# Autodesk Inventor assembly: Storage System Assembly
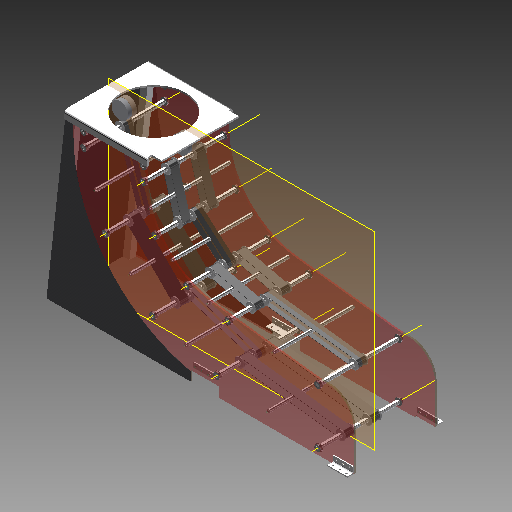
[picture p0: Inventor's stored thumbnail of the model, 512x512]
Saved by Autodesk Inventor 2019.4 (Build 234330000, 330)
## iProperties
Created: 2020-01-11
Part Number: Storage System Assembly
Document SubType Name: Assembly
Designer: admin
Mass: 9233.81 g
Surface Area: 26399.2 cm^2
Volume: 4839.78 cm^3
Density: 1.9079 g/cm^3
Author: admin
## Documents named in this file (23)
- C:\Users\Mark\Desktop\7738 Helion Engineering\7738-2020\Storage system\Storage System Assembly.iam
- C:\Users\Mark\Desktop\7738 Helion Engineering\7738-2020\Storage system\Turret Base Plate.ipt
- C:\Users\Mark\Desktop\7738 Helion Engineering\7738-2020\Storage system\Storage Side Plate.ipt
- C:\Users\Mark\Desktop\7738 Helion Engineering\7738-2020\CAD\Gearbox\F6800.ipt
- C:\Users\Mark\Desktop\7738 Helion Engineering\7738-2020\Storage system\Storage System Assembly\Design Accelerator\Synchronous Belts Transmission1.iam
- C:\Users\Mark\Desktop\7738 Helion Engineering\7738-2020\Storage system\Storage System Assembly\Design Accelerator\Synchronous Belts Transmission2.iam
- C:\Users\Mark\Desktop\7738 Helion Engineering\7738-2020\Storage system\Storage System Assembly\Design Accelerator\Synchronous Belts Transmission3.iam
- C:\Users\Mark\Desktop\7738 Helion Engineering\7738-2020\Storage system\Storage System Assembly\Design Accelerator\Synchronous Belts Transmission5.iam
- C:\Users\Mark\Desktop\7738 Helion Engineering\7738-2020\Storage system\Storage System Assembly\Design Accelerator\Synchronous Belts Transmission6.iam
- C:\Users\Mark\Desktop\7738 Helion Engineering\7738-2020\Storage system\Storage System Assembly\Design Accelerator\Synchronous Belts Transmission7.iam
- C:\Users\Mark\Desktop\7738 Helion Engineering\7738-2020\Storage system\Storage System Assembly\Design Accelerator\Synchronous Belts Transmission8.iam
- C:\Users\Mark\Desktop\7738 Helion Engineering\7738-2020\Storage system\Storage System Assembly\Design Accelerator\Synchronous Belts Transmission9.iam
- C:\Users\Mark\Desktop\7738 Helion Engineering\7738-2020\Storage system\Complaint Wheel.ipt
- C:\Users\Mark\Desktop\7738 Helion Engineering\7738-2020\Storage system\Belt Axle.ipt
- C:\Users\Mark\Desktop\7738 Helion Engineering\7738-2020\Storage system\Storage System Assembly\Design Accelerator\Synchronous Belts Transmission4.iam
- C:\Users\Mark\Desktop\7738 Helion Engineering\7738-2020\Storage system\Storage System Assembly\Design Accelerator\Synchronous Belts Transmission10.iam
- C:\Users\Mark\Desktop\7738 Helion Engineering\7738-2020\Storage system\Storage System Assembly\Design Accelerator\Synchronous Belts Transmission11.iam
- C:\Users\Mark\Desktop\7738 Helion Engineering\7738-2020\Storage system\Storage System Assembly\Design Accelerator\Synchronous Belts Transmission12.iam
- C:\Users\Mark\Desktop\7738 Helion Engineering\7738-2020\Storage system\Storage Plate Spacer.ipt
- C:\Users\Mark\Desktop\7738 Helion Engineering\7738-2020\Storage system\PC Plate Bracket.ipt
- C:\Users\Mark\Desktop\7738 Helion Engineering\7738-2020\Storage system\Turret Support Extrusion.ipt
- C:\Users\Mark\Desktop\7738 Helion Engineering\7738-2020\Storage system\Back PC Cover.ipt
- C:\Users\Mark\Desktop\7738 Helion Engineering\7738-2020\Storage system\Side CFRP Cover.ipt
## Components (70 placed, 11 different names)
1. Turret Base Plate:1 — Mate:1, Mate:3, Mate:4, Flush:1, Mate:5, Mate:8, Mate:9, Angle:1, Mate:107, Mate:108, Mate:110
2. Storage Side Plate:1 — Mate:1, Mate:7, Mate:8, Mate:10, Mate:11, Mate:12, Mate:13, Mate:14, Mate:15, Mate:16, Mate:17, Mate:18, Mate:19, Mate:20, Mate:21, Mate:22, Mate:23, Mate:24, Mate:25, Mate:26, Mate:27, Mate:28, Mate:29, Mate:30, Mate:31, Mate:32, Mate:33, Symmetry:1, Mate:75, Mate:93, Mate:94, Mate:95, Mate:96, Mate:97, Mate:98, Mate:99, Mate:100, Mate:101, Flush:4, Mate:102, Mate:105, Flush:6, Flush:7, Mate:107, Mate:111, Flush:11, Mate:114, Mate:115, Flush:12, Flush:13
3. Storage Side Plate:2 — Mate:5, Mate:7, Mate:9, Symmetry:1, Mate:41, Mate:42, Mate:43, Mate:44, Mate:45, Mate:46, Mate:47, Mate:48, Mate:49, Mate:50, Mate:51, Mate:52, Mate:53, Mate:54, Mate:55, Mate:56, Mate:57, Mate:58, Mate:59, Mate:60, Mate:61, Mate:62, Mate:63, Mate:64, Mate:85, Mate:86, Mate:87, Mate:88, Mate:89, Mate:90, Mate:91, Mate:92, Mate:103, Mate:104, Flush:5, Mate:106, Flush:8, Flush:9, Mate:109, Flush:10, Mate:113, Mate:116, Flush:14, Flush:15
4. Synchronous Belts Transmission:1 [sub-assembly] — Mate:66
5. Synchronous Belts Transmission:2 [sub-assembly]
6. Synchronous Belts Transmission:3 [sub-assembly]
7. Synchronous Belts Transmission:4 [sub-assembly]
8. Synchronous Belts Transmission:5 [sub-assembly]
9. Synchronous Belts Transmission:6 [sub-assembly]
10. Synchronous Belts Transmission:7 [sub-assembly]
11. Synchronous Belts Transmission:8 [sub-assembly]
12. F6800:11 — Mate:30, Mate:32, Mate:34
13. F6800:12 — Mate:31, Mate:33, Mate:39
14. Complaint Wheel:1 — Mate:34, Mate:35, Mate:36, Flush:3
15. Complaint Wheel:2 — Mate:35, Mate:36, Mate:40
16. Complaint Wheel:3 — Flush:3
17. Complaint Wheel:4 — Mate:39
18. Synchronous Belts Transmission:9 [sub-assembly]
19. Synchronous Belts Transmission:10 [sub-assembly]
20. Synchronous Belts Transmission:11 [sub-assembly]
21. Synchronous Belts Transmission:12 [sub-assembly]
22. Storage Plate Spacer:1 — Mate:85, Mate:93
23. Storage Plate Spacer:2 — Mate:89, Mate:100
24. Storage Plate Spacer:3 — Mate:90, Mate:99
25. Storage Plate Spacer:4 — Mate:91, Mate:98
26. Storage Plate Spacer:5 — Mate:92, Mate:97
27. Storage Plate Spacer:6 — Mate:88, Mate:96
28. Storage Plate Spacer:7 — Mate:87, Mate:95
29. Storage Plate Spacer:8 — Mate:86, Mate:94
30. PC Plate Bracket:1 — Mate:101, Flush:4, Mate:102
31. PC Plate Bracket:2 — Mate:103, Mate:104, Flush:5
32. PC Plate Bracket:3 — Mate:105, Flush:6, Flush:7
33. PC Plate Bracket:4 — Mate:106, Flush:8, Flush:9
34. Turret Support Extrusion:1 — Mate:108, Mate:109, Flush:10, Mate:112
35. Turret Support Extrusion:2 — Mate:110, Mate:111, Flush:11
36. Back PC Cover:1 — Mate:112, Mate:113, Mate:114
37. Side CFRP Cover:1 — Mate:115, Flush:12, Flush:13
38. Side CFRP Cover:2 — Mate:116, Flush:14, Flush:15
39. Belt Axle:10 — Mate:74, Mate:84
40. Belt Axle:9 — Mate:73, Mate:83
41. Belt Axle:8 — Mate:72, Mate:82
42. Belt Axle:7 — Mate:71, Mate:81
43. Belt Axle:6 — Mate:70, Mate:80
44. Belt Axle:5 — Mate:69, Mate:75
45. Belt Axle:4 — Mate:68, Mate:76
46. Belt Axle:3 — Mate:67, Mate:77
47. Belt Axle:2 — Mate:66, Mate:78
48. Belt Axle:1 — Mate:65, Mate:79
49. F6800:10 — Mate:19, Mate:25, Mate:70, Mate:80
50. F6800:9 — Mate:18, Mate:26, Mate:71, Mate:81
51. F6800:7 — Mate:16, Mate:28, Mate:73, Mate:83
52. F6800:8 — Mate:17, Mate:27, Mate:72, Mate:82
53. F6800:6 — Mate:15, Mate:29, Mate:74, Mate:84
54. F6800:5 — Mate:14, Mate:24, Mate:69
55. F6800:4 — Mate:13, Mate:23, Mate:68, Mate:76
56. F6800:3 — Mate:12, Mate:22, Mate:67, Mate:77
57. F6800:2 — Mate:11, Mate:21, Mate:78
58. F6800:1 — Mate:10, Mate:20, Mate:65, Mate:79
59. F6800:24 — Mate:52, Mate:64
60. F6800:23 — Mate:51, Mate:63
61. F6800:22 — Mate:49, Mate:61
62. F6800:21 — Mate:50, Mate:62
63. F6800:20 — Mate:48, Mate:60
64. F6800:19 — Mate:47, Mate:59
65. F6800:18 — Mate:46, Mate:57
66. F6800:17 — Mate:45, Mate:58
67. F6800:16 — Mate:44, Mate:55
68. F6800:15 — Mate:42, Mate:53
69. F6800:13 — Mate:41, Mate:54
70. F6800:14 — Mate:43, Mate:56
## Relationships (130: Mate 114, Flush 14, Angle 1, Symmetry 1)
- Mate:1: Turret Base Plate:1 ↔ Storage Side Plate:1
- Mate:3: Turret Base Plate:1
- Mate:4: Turret Base Plate:1
- Flush:1: Turret Base Plate:1
- Mate:5: Turret Base Plate:1 ↔ Storage Side Plate:2
- Mate:7: Storage Side Plate:1 ↔ Storage Side Plate:2
- Mate:8 (3 mm): Turret Base Plate:1 ↔ Storage Side Plate:1
- Mate:9 (3 mm): Turret Base Plate:1 ↔ Storage Side Plate:2
- Mate:10: Storage Side Plate:1 ↔ F6800:1
- Mate:11: Storage Side Plate:1 ↔ F6800:2
- Mate:12: Storage Side Plate:1 ↔ F6800:3
- Mate:13: Storage Side Plate:1 ↔ F6800:4
- Mate:14: Storage Side Plate:1 ↔ F6800:5
- Mate:15: Storage Side Plate:1 ↔ F6800:6
- Mate:16: Storage Side Plate:1 ↔ F6800:7
- Mate:17: Storage Side Plate:1 ↔ F6800:8
- Mate:18: Storage Side Plate:1 ↔ F6800:9
- Mate:19: Storage Side Plate:1 ↔ F6800:10
- Mate:20 (0.2 mm): Storage Side Plate:1 ↔ F6800:1
- Mate:21 (0.2 mm): Storage Side Plate:1 ↔ F6800:2
- Mate:22 (0.2 mm): Storage Side Plate:1 ↔ F6800:3
- Mate:23 (0.2 mm): Storage Side Plate:1 ↔ F6800:4
- Mate:24 (0.2 mm): Storage Side Plate:1 ↔ F6800:5
- Mate:25 (0.2 mm): Storage Side Plate:1 ↔ F6800:10
- Mate:26 (0.2 mm): Storage Side Plate:1 ↔ F6800:9
- Mate:27 (0.2 mm): Storage Side Plate:1 ↔ F6800:8
- Mate:28 (0.2 mm): Storage Side Plate:1 ↔ F6800:7
- Mate:29 (0.2 mm): Storage Side Plate:1 ↔ F6800:6
- Angle:1 (180 deg): Turret Base Plate:1
- Mate:30: Storage Side Plate:1 ↔ F6800:11
- Mate:31: Storage Side Plate:1 ↔ F6800:12
- Mate:32 (0.2 mm): Storage Side Plate:1 ↔ F6800:11
- Mate:33 (0.2 mm): Storage Side Plate:1 ↔ F6800:12
- Mate:34: F6800:11 ↔ Complaint Wheel:1
- Mate:35: Complaint Wheel:1 ↔ Complaint Wheel:2
- Mate:36 (1 mm): Complaint Wheel:1 ↔ Complaint Wheel:2
- [Mate]: Complaint Wheel:3 ↔ Complaint Wheel:4
- [Mate] (1 mm): Complaint Wheel:3 ↔ Complaint Wheel:4
- Mate:39: F6800:12 ↔ Complaint Wheel:4
- Flush:3: Complaint Wheel:1 ↔ Complaint Wheel:3
- Symmetry:1: Storage Side Plate:1 ↔ Storage Side Plate:2
- Mate:40 (0.5 mm): Complaint Wheel:2
- Mate:41: Storage Side Plate:2 ↔ F6800:13
- Mate:42: Storage Side Plate:2 ↔ F6800:15
- Mate:43: Storage Side Plate:2 ↔ F6800:14
- Mate:44: Storage Side Plate:2 ↔ F6800:16
- Mate:45: Storage Side Plate:2 ↔ F6800:17
- Mate:46: Storage Side Plate:2 ↔ F6800:18
- Mate:47: Storage Side Plate:2 ↔ F6800:19
- Mate:48: Storage Side Plate:2 ↔ F6800:20
- Mate:49: Storage Side Plate:2 ↔ F6800:22
- Mate:50: Storage Side Plate:2 ↔ F6800:21
- Mate:51: Storage Side Plate:2 ↔ F6800:23
- Mate:52: Storage Side Plate:2 ↔ F6800:24
- Mate:53 (0.2 mm): Storage Side Plate:2 ↔ F6800:15
- Mate:54 (0.2 mm): Storage Side Plate:2 ↔ F6800:13
- Mate:55 (0.2 mm): Storage Side Plate:2 ↔ F6800:16
- Mate:56 (0.2 mm): Storage Side Plate:2 ↔ F6800:14
- Mate:57 (0.2 mm): Storage Side Plate:2 ↔ F6800:18
- Mate:58 (0.2 mm): Storage Side Plate:2 ↔ F6800:17
- Mate:59 (0.2 mm): Storage Side Plate:2 ↔ F6800:19
- Mate:60 (0.2 mm): Storage Side Plate:2 ↔ F6800:20
- Mate:61 (0.2 mm): Storage Side Plate:2 ↔ F6800:22
- Mate:62 (0.2 mm): Storage Side Plate:2 ↔ F6800:21
- Mate:63 (0.2 mm): Storage Side Plate:2 ↔ F6800:23
- Mate:64 (0.2 mm): Storage Side Plate:2 ↔ F6800:24
- Mate:65: Belt Axle:1 ↔ F6800:1
- Mate:66: Synchronous Belts Transmission:1 ↔ Belt Axle:2
- Mate:67: Belt Axle:3 ↔ F6800:3
- Mate:68: Belt Axle:4 ↔ F6800:4
- Mate:69: Belt Axle:5 ↔ F6800:5
- Mate:70: Belt Axle:6 ↔ F6800:10
- Mate:71: Belt Axle:7 ↔ F6800:9
- Mate:72: Belt Axle:8 ↔ F6800:8
- Mate:73: Belt Axle:9 ↔ F6800:7
- Mate:74: Belt Axle:10 ↔ F6800:6
- Mate:75 (0.2 mm): Storage Side Plate:1 ↔ Belt Axle:5
- Mate:76 (0.2 mm): Belt Axle:4 ↔ F6800:4
- Mate:77 (0.2 mm): Belt Axle:3 ↔ F6800:3
- Mate:78 (0.2 mm): Belt Axle:2 ↔ F6800:2
- Mate:79 (0.2 mm): Belt Axle:1 ↔ F6800:1
- Mate:80 (0.2 mm): Belt Axle:6 ↔ F6800:10
- Mate:81 (0.2 mm): Belt Axle:7 ↔ F6800:9
- Mate:82 (0.2 mm): Belt Axle:8 ↔ F6800:8
- Mate:83 (0.2 mm): Belt Axle:9 ↔ F6800:7
- Mate:84 (0.2 mm): Belt Axle:10 ↔ F6800:6
- Mate:85: Storage Side Plate:2 ↔ Storage Plate Spacer:1
- Mate:86: Storage Side Plate:2 ↔ Storage Plate Spacer:8
- Mate:87: Storage Side Plate:2 ↔ Storage Plate Spacer:7
- Mate:88: Storage Side Plate:2 ↔ Storage Plate Spacer:6
- Mate:89: Storage Side Plate:2 ↔ Storage Plate Spacer:2
- Mate:90: Storage Side Plate:2 ↔ Storage Plate Spacer:3
- Mate:91: Storage Side Plate:2 ↔ Storage Plate Spacer:4
- Mate:92: Storage Side Plate:2 ↔ Storage Plate Spacer:5
- Mate:93 (0.2 mm): Storage Side Plate:1 ↔ Storage Plate Spacer:1
- Mate:94 (0.2 mm): Storage Side Plate:1 ↔ Storage Plate Spacer:8
- Mate:95 (0.2 mm): Storage Side Plate:1 ↔ Storage Plate Spacer:7
- Mate:96 (0.2 mm): Storage Side Plate:1 ↔ Storage Plate Spacer:6
- Mate:97 (0.2 mm): Storage Side Plate:1 ↔ Storage Plate Spacer:5
- Mate:98 (0.2 mm): Storage Side Plate:1 ↔ Storage Plate Spacer:4
- Mate:99 (0.2 mm): Storage Side Plate:1 ↔ Storage Plate Spacer:3
- Mate:100 (0.2 mm): Storage Side Plate:1 ↔ Storage Plate Spacer:2
- Mate:101: Storage Side Plate:1 ↔ PC Plate Bracket:1
- Flush:4: Storage Side Plate:1 ↔ PC Plate Bracket:1
- Mate:102 (3 mm): Storage Side Plate:1 ↔ PC Plate Bracket:1
- Mate:103: Storage Side Plate:2 ↔ PC Plate Bracket:2
- Mate:104 (3 mm): Storage Side Plate:2 ↔ PC Plate Bracket:2
- Flush:5: Storage Side Plate:2 ↔ PC Plate Bracket:2
- Mate:105: Storage Side Plate:1 ↔ PC Plate Bracket:3
- Flush:6: Storage Side Plate:1 ↔ PC Plate Bracket:3
- Flush:7: Storage Side Plate:1 ↔ PC Plate Bracket:3
- Mate:106: Storage Side Plate:2 ↔ PC Plate Bracket:4
- Flush:8: Storage Side Plate:2 ↔ PC Plate Bracket:4
- Flush:9: Storage Side Plate:2 ↔ PC Plate Bracket:4
- Mate:107: Turret Base Plate:1 ↔ Storage Side Plate:1
- Mate:108: Turret Base Plate:1 ↔ Turret Support Extrusion:1
- Mate:109: Storage Side Plate:2 ↔ Turret Support Extrusion:1
- Flush:10 (5 mm): Storage Side Plate:2 ↔ Turret Support Extrusion:1
- Mate:110: Turret Base Plate:1 ↔ Turret Support Extrusion:2
- Mate:111: Storage Side Plate:1 ↔ Turret Support Extrusion:2
- Flush:11 (5 mm): Storage Side Plate:1 ↔ Turret Support Extrusion:2
- Mate:112: Turret Support Extrusion:1 ↔ Back PC Cover:1
- Mate:113 (1 mm): Storage Side Plate:2 ↔ Back PC Cover:1
- Mate:114: Storage Side Plate:1 ↔ Back PC Cover:1
- Mate:115: Storage Side Plate:1 ↔ Side CFRP Cover:1
- Flush:12: Storage Side Plate:1 ↔ Side CFRP Cover:1
- Flush:13: Storage Side Plate:1 ↔ Side CFRP Cover:1
- Mate:116: Storage Side Plate:2 ↔ Side CFRP Cover:2
- Flush:14: Storage Side Plate:2 ↔ Side CFRP Cover:2
- Flush:15: Storage Side Plate:2 ↔ Side CFRP Cover:2
## Named parameters: d40_d38 = 0 mm, d41_d39 = 1 mm
